# Autodesk Inventor assembly: plotter_try_2
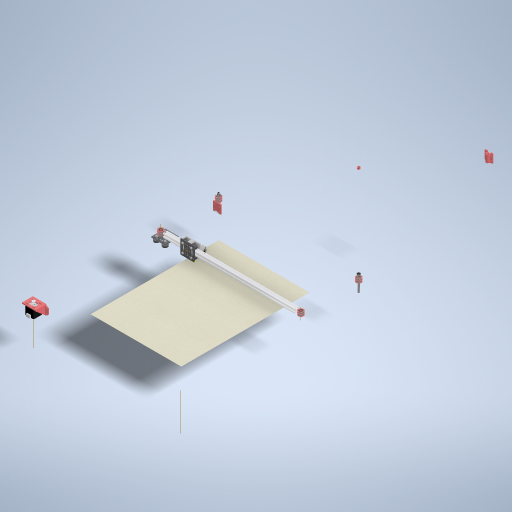
[picture p0: Inventor's stored thumbnail of the model, 512x512]
Saved by Autodesk Inventor 2023 (Build 270158000, 158)
## iProperties
RuleStatus: InUse
Created: 2023-08-15
Part Number: plotter_try_2
Document SubType Name: Assembly
Designer: Felix
_SolveAssemblyDoc: Frame Generator Solve Assembly
_Version: 15.0.0
Author: Felix
## Documents named in this file (20)
- D:\Programmieren\PineapplePenPlotter\Inventor\plotter_try_3.iam
- D:\Programmieren\PineapplePenPlotter\Inventor\PaperA2.ipt
- D:\Programmieren\PineapplePenPlotter\Inventor\plotter_try_2\Frame2.ipt
- D:\Programmieren\PineapplePenPlotter\Inventor\plotter_try_2\Frame\Frame 1692119975215.iam
- D:\Programmieren\PineapplePenPlotter\Inventor\StoreBought\4022_20220624140806_V-Slot Gantry Kit - 20mm.iam
- D:\Programmieren\PineapplePenPlotter\Inventor\try_3\YAxisFrame.ipt
- D:\Programmieren\PineapplePenPlotter\Inventor\plotter_try_3\Frame\1692309134113.ipt
- D:\Programmieren\PineapplePenPlotter\Inventor\try_3\RollerSmall.iam
- D:\Programmieren\PineapplePenPlotter\Inventor\try_3\AxisLocations.ipt
- D:\Programmieren\PineapplePenPlotter\Inventor\try_3\AxleHolder.ipt
- C:\Users\Felix\Documents\Inventor\Content Center Files\R2023\en-US\AS 1111\AS 1111 - M8 x 70.ipt
- D:\Programmieren\PineapplePenPlotter\Inventor\try_3\M8Spacer.ipt
- D:\Programmieren\PineapplePenPlotter\Inventor\try_3\RollerSmallNoSpacer.iam
- D:\Programmieren\PineapplePenPlotter\Inventor\try_3\SpacerM8.ipt
- C:\Users\Felix\Documents\Inventor\Content Center Files\R2023\en-US\DIN 934\DIN 934 - M8 x 1,25.ipt
- D:\Programmieren\PineapplePenPlotter\Inventor\StoreBought\GT2_16T.ipt
- D:\Programmieren\PineapplePenPlotter\Inventor\steppeSquare.ipt
- D:\Programmieren\PineapplePenPlotter\Inventor\try_3\MotorBracketV2.ipt
- D:\Programmieren\PineapplePenPlotter\Inventor\try_3\Penholder.iam
- D:\Programmieren\PineapplePenPlotter\Inventor\beltTest.ipt
## Components (30 placed, 19 different names)
1. PaperA2:1 — Flush:1, Mate:2, Angle:1, Flush:11, Flush:20, Angle:4, Angle:5, Flush:27, Angle:11, Flush:45
2. Frame2:1 — Flush:1
3. YAxisFrame:1 — Flush:8, Flush:9
4. Frame 1692119975215:1 [sub-assembly] — Mate:1, Flush:2, Flush:3, Mate:3, Flush:19, Flush:24, Flush:30
5. 4022_20220624140806_V-Slot Gantry Kit - 20mm:1 [sub-assembly] — Mate:1, Flush:2, Flush:4, Flush:9, Flush:10, Mate:11, Mate:12, Mate:14, Mate:40
6. 4022_20220624140806_V-Slot Gantry Kit - 20mm:2 [sub-assembly] — Flush:3, Mate:3, Flush:4, Flush:8, Flush:19, Mate:13, Mate:39
7. - 538,9:1 — Flush:10, Mate:11, Mate:12, Mate:37, Flush:39, Mate:38, Mate:39
8. RollerSmall:1 [sub-assembly] — Mate:18, Flush:21
9. AxisLocations:1 — Flush:20, Mate:16, Mate:17, Flush:26, Mate:21, Mate:22, Mate:31, Mate:32
10. RollerSmall:2 [sub-assembly] — Flush:22, Mate:19
11. AxleHolder:1 — Flush:27, Mate:24
12. AS 1111 - Metric M8 x 70:1 — Mate:20, Flush:24, Mate:23, Mate:25, Mate:26, Mate:28, Mate:29
13. M8Spacer:1 — Mate:23, Mate:24
14. RollerSmallNoSpacer:1 [sub-assembly] — Mate:25, Mate:27, Flush:28
15. SpacerM8:1 — Mate:26, Mate:27
16. RollerSmallNoSpacer:2 [sub-assembly] — Mate:28, Flush:29, Mate:30
17. DIN 934 - replaced by DIN EN 24032/28673/28674 M8:1 — Mate:29, Mate:30
18. GT2_16T:1 — Mate:33, Mate:34, Mate:35, Mate:36
19. steppeSquare:1 — Mate:35, Mate:36, Angle:10
20. MotorBracketV2:1 — Flush:30
21. Penholder:1 [sub-assembly] — Flush:39, Mate:38, Mate:40
22. RollerSmall:3 [sub-assembly] — Flush:41, Mate:41
23. RollerSmall:4 [sub-assembly] — Mate:42, Flush:42
24. AxleHolder:2 — Mate:44
25. AS 1111 - Metric M8 x 70:2 — Mate:43, Mate:45, Mate:46, Mate:47
26. M8Spacer:2 — Mate:44, Mate:45
27. RollerSmallNoSpacer:3 [sub-assembly] — Flush:43, Mate:46
28. RollerSmallNoSpacer:4 [sub-assembly] — Flush:44, Mate:47, Mate:48
29. DIN 934 - replaced by DIN EN 24032/28673/28674 M8:2 — Mate:48
30. beltTest:1 — Flush:45
## Relationships (75: Mate 40, Flush 26, Angle 9)
- Flush:1: PaperA2:1 ↔ Frame2:1
- Mate:1: Frame 1692119975215:1 ↔ 4022_20220624140806_V-Slot Gantry Kit - 20mm:1
- Flush:2: Frame 1692119975215:1 ↔ 4022_20220624140806_V-Slot Gantry Kit - 20mm:1
- Mate:2: PaperA2:1
- Angle:1 (0 deg): PaperA2:1
- Flush:3: Frame 1692119975215:1 ↔ 4022_20220624140806_V-Slot Gantry Kit - 20mm:2
- Mate:3: Frame 1692119975215:1 ↔ 4022_20220624140806_V-Slot Gantry Kit - 20mm:2
- Flush:4: 4022_20220624140806_V-Slot Gantry Kit - 20mm:1 ↔ 4022_20220624140806_V-Slot Gantry Kit - 20mm:2
- Flush:8: YAxisFrame:1 ↔ 4022_20220624140806_V-Slot Gantry Kit - 20mm:2
- Flush:9: YAxisFrame:1 ↔ 4022_20220624140806_V-Slot Gantry Kit - 20mm:1
- Flush:10: 4022_20220624140806_V-Slot Gantry Kit - 20mm:1 ↔ - 538,9:1
- Mate:11 (-10 mm): 4022_20220624140806_V-Slot Gantry Kit - 20mm:1 ↔ - 538,9:1
- Mate:12: 4022_20220624140806_V-Slot Gantry Kit - 20mm:1 ↔ - 538,9:1
- Flush:11 (-49.5 mm): PaperA2:1
- Flush:12 (-9 mm)
- Flush:19: Frame 1692119975215:1 ↔ 4022_20220624140806_V-Slot Gantry Kit - 20mm:2
- Mate:13: 4022_20220624140806_V-Slot Gantry Kit - 20mm:2
- Mate:14: 4022_20220624140806_V-Slot Gantry Kit - 20mm:1
- Flush:20: PaperA2:1 ↔ AxisLocations:1
- Mate:16: AxisLocations:1
- Angle:4 (0 deg): PaperA2:1
- Mate:17: AxisLocations:1
- Angle:5 (0 deg): PaperA2:1
- Mate:18: RollerSmall:1
- Flush:21 (-3.5 mm): RollerSmall:1
- Flush:22 (-3.5 mm): RollerSmall:2
- Mate:19: RollerSmall:2
- Mate:20: AS 1111 - Metric M8 x 70:1
- Flush:24 (1 mm): Frame 1692119975215:1 ↔ AS 1111 - Metric M8 x 70:1
- Flush:26: AxisLocations:1
- Mate:21: AxisLocations:1
- Angle:6 (0 deg)
- Mate:22: AxisLocations:1
- Angle:7 (0 deg)
- Flush:27 (-1 mm): PaperA2:1 ↔ AxleHolder:1
- Mate:23: AS 1111 - Metric M8 x 70:1 ↔ M8Spacer:1
- Mate:24: AxleHolder:1 ↔ M8Spacer:1
- Mate:25: AS 1111 - Metric M8 x 70:1 ↔ RollerSmallNoSpacer:1
- Mate:26: AS 1111 - Metric M8 x 70:1 ↔ SpacerM8:1
- Mate:27: RollerSmallNoSpacer:1 ↔ SpacerM8:1
- Flush:28 (-3.5 mm): RollerSmallNoSpacer:1
- Mate:28: AS 1111 - Metric M8 x 70:1 ↔ RollerSmallNoSpacer:2
- Flush:29 (-3.5 mm): RollerSmallNoSpacer:2
- Mate:29: AS 1111 - Metric M8 x 70:1 ↔ DIN 934 - replaced by DIN EN 24032/28673/28674 M8:1
- Mate:30: RollerSmallNoSpacer:2 ↔ DIN 934 - replaced by DIN EN 24032/28673/28674 M8:1
- Mate:31: AxisLocations:1
- Angle:8 (0 deg)
- Mate:32: AxisLocations:1
- Angle:9 (0 deg)
- Mate:33: GT2_16T:1
- Mate:34 (3.5 mm): GT2_16T:1
- Mate:35: GT2_16T:1 ↔ steppeSquare:1
- Mate:36 (0.5 mm): GT2_16T:1 ↔ steppeSquare:1
- Angle:10 (0 deg): steppeSquare:1
- Flush:30: Frame 1692119975215:1 ↔ MotorBracketV2:1
- Mate:37: - 538,9:1
- Angle:11 (0 deg): PaperA2:1
- Flush:39: - 538,9:1 ↔ Penholder:1
- Mate:38 (-10 mm): - 538,9:1 ↔ Penholder:1
- Mate:39: 4022_20220624140806_V-Slot Gantry Kit - 20mm:2 ↔ - 538,9:1
- Mate:40: 4022_20220624140806_V-Slot Gantry Kit - 20mm:1 ↔ Penholder:1
- Flush:40 (-9 mm)
- Flush:41 (-3.5 mm): RollerSmall:3
- Mate:41: RollerSmall:3
- Mate:42: RollerSmall:4
- Flush:42 (-3.5 mm): RollerSmall:4
- Mate:43: AS 1111 - Metric M8 x 70:2
- Mate:44: AxleHolder:2 ↔ M8Spacer:2
- Mate:45: AS 1111 - Metric M8 x 70:2 ↔ M8Spacer:2
- Flush:43 (-3.5 mm): RollerSmallNoSpacer:3
- Mate:46: AS 1111 - Metric M8 x 70:2 ↔ RollerSmallNoSpacer:3
- Flush:44 (-3.5 mm): RollerSmallNoSpacer:4
- Mate:47: AS 1111 - Metric M8 x 70:2 ↔ RollerSmallNoSpacer:4
- Mate:48: RollerSmallNoSpacer:4 ↔ DIN 934 - replaced by DIN EN 24032/28673/28674 M8:2
- Flush:45: PaperA2:1 ↔ beltTest:1
## Named parameters: ROLLER_SPACING = 2 mm, BELT_THICKNESS = 1.5 mm, RIGHT_MOTOR_HEIGHT = 50 mm
